# Autodesk Inventor assembly: Drivetrain2
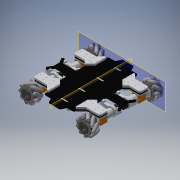
[picture p0: Inventor's stored thumbnail of the model, 180x180]
Saved by Autodesk Inventor 2018 (Build 220112000, 112)
## iProperties
Created: 2018-09-24
Part Number: Drivetrain2
Document SubType Name: Assembly
Designer: anirudh
Author: anirudh
## Documents named in this file (9)
- C:\Users\anirudh\Documents\MARS Fund\Jetson\JetsonCar\Drivetrain\Drivetrain2.iam
- C:\Users\anirudh\Documents\MARS Fund\Jetson\JetsonCar\Drivetrain\Acrylic Drivetrain Base - 1.ipt
- C:\Users\anirudh\Documents\MARS Fund\Jetson\JetsonCar\Drivetrain\BottomMotorSuspension.ipt
- C:\Users\anirudh\Documents\MARS Fund\Jetson\JetsonCar\Drivetrain\TopMotorSuspension.ipt
- C:\Users\anirudh\Documents\MARS Fund\Jetson\JetsonCar\Drivetrain\ExpansionHubREV.ipt
- C:\Users\anirudh\Documents\MARS Fund\Jetson\JetsonCar\Drivetrain\RightMotorBracket.ipt
- C:\Users\anirudh\Documents\MARS Fund\Jetson\JetsonCar\Drivetrain\LeftMotorBracket.ipt
- C:\Users\anirudh\Documents\MARS Fund\Jetson\JetsonCar\Drivetrain\Wheel Assemblies\RightWheelAssembly.iam
- C:\Users\anirudh\Documents\MARS Fund\Jetson\JetsonCar\Drivetrain\Wheel Assemblies\LeftWheelAssembly.iam
## Components (21 placed, 8 different names)
1. Acrylic Drivetrain Base - 1:1 — Symmetry:2
2. BottomMotorSuspension:1 — Insert:10
3. BottomMotorSuspension:2 — Insert:11
4. BottomMotorSuspension:3 — Insert:13
5. BottomMotorSuspension:4 — Insert:12
6. TopMotorSuspension:1 — Symmetry:2
7. TopMotorSuspension:2
8. TopMotorSuspension:3
9. TopMotorSuspension:4
10. ExpansionHubREV:1
11. ExpansionHubREV:2 — Flush:9
12. ExpansionHubREV:3
13. ExpansionHubREV:4 — Flush:9
14. RightMotorBracket:1
15. RightMotorBracket:2
16. LeftMotorBracket:1
17. LeftMotorBracket:2
18. RightWheelAssembly:1 [sub-assembly] — Insert:11, Symmetry:1
19. RightWheelAssembly:2 [sub-assembly] — Insert:10
20. LeftWheelAssembly:1 [sub-assembly] — Insert:13
21. LeftWheelAssembly:2 [sub-assembly] — Insert:12, Symmetry:1
## Relationships (7: Insert 4, Symmetry 2, Flush 1)
- Flush:9: ExpansionHubREV:2 ↔ ExpansionHubREV:4
- Insert:10: BottomMotorSuspension:1 ↔ RightWheelAssembly:2
- Insert:11: BottomMotorSuspension:2 ↔ RightWheelAssembly:1
- Insert:12: BottomMotorSuspension:4 ↔ LeftWheelAssembly:2
- Insert:13: BottomMotorSuspension:3 ↔ LeftWheelAssembly:1
- Symmetry:1: RightWheelAssembly:1 ↔ LeftWheelAssembly:2
- Symmetry:2: Acrylic Drivetrain Base - 1:1 ↔ TopMotorSuspension:1
